# Autodesk Inventor assembly: MarcoSuperior
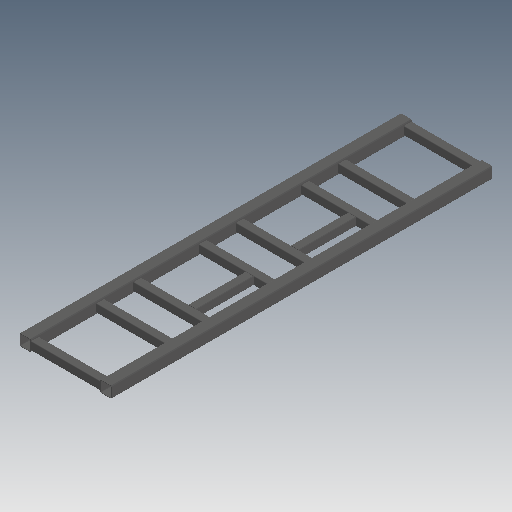
[picture p0: Inventor's stored thumbnail of the model, 512x512]
Saved by Autodesk Inventor 2021 (Build 250183000, 183)
## iProperties
_SolveAssemblyDoc: Frame Generator Solve Assembly
_Version: 25.0.0
Created: 2021-05-05
Part Number: MarcoSuperior
Document SubType Name: Assembly
Designer: Santiago Suárez
Mass: 41792.5 g
Surface Area: 40236.4 cm^2
Volume: 5244.14 cm^3
Density: 7.96936 g/cm^3
Author: Santiago Suárez
## Documents named in this file (9)
- C:\Users\Santiago Suárez\Documents\GitHub\Dis.-Mecatronico-E6\inventor proyecto\MarcoSuperior.iam
- C:\Users\Santiago Suárez\Documents\GitHub\Dis.-Mecatronico-E6\inventor proyecto\Marco central.ipt
- C:\Users\Santiago Suárez\Documents\GitHub\Dis.-Mecatronico-E6\inventor proyecto\MarcoSuperior\Frame\MarcoSuperior.iam
- C:\Users\Santiago Suárez\Documents\GitHub\Dis.-Mecatronico-E6\inventor proyecto\MarcoSuperior\AIP\FEA\dn1qp8i5c.fins
- C:\Users\Santiago Suárez\Documents\GitHub\Dis.-Mecatronico-E6\inventor proyecto\MarcoSuperior\AIP\FEA\dn1qp8i5c.fsat
- C:\Users\Santiago Suárez\Documents\GitHub\Dis.-Mecatronico-E6\inventor proyecto\MarcoSuperior\AIP\FEA\dn1qp8i68.ftes
- C:\Users\Santiago Suárez\Documents\GitHub\Dis.-Mecatronico-E6\inventor proyecto\MarcoSuperior\AIP\FEA\dn1qp8i68.fwiz
- C:\Users\Santiago Suárez\Documents\GitHub\Dis.-Mecatronico-E6\inventor proyecto\MarcoSuperior\AIP\FEA\dn1qp8kv4.fmsh
- C:\Users\Santiago Suárez\Documents\GitHub\Dis.-Mecatronico-E6\inventor proyecto\MarcoSuperior\AIP\FEA\dn1qp8kv5.fres
## Components (2 placed, 2 different names)
1. Marco central:1
2. MarcoSuperior:1 [sub-assembly]
## Named parameters: sa_1 = 981, sa_0 = 69000, sa_2 = 69000, sa_3 = 69000, sa_4 = 69000, sa_5 = 69000, sa_6 = 69000, sa_7 = 69000, sa_8 = 69000
note: some values were not read from the file. Shown as the stored number, unit unknown: "sa_1", "sa_0", "sa_2", "sa_3", "sa_4", "sa_5", "sa_6", "sa_7", "sa_8".
